# Autodesk Inventor assembly: ASY MSC 100.3 ROСKET NOSE
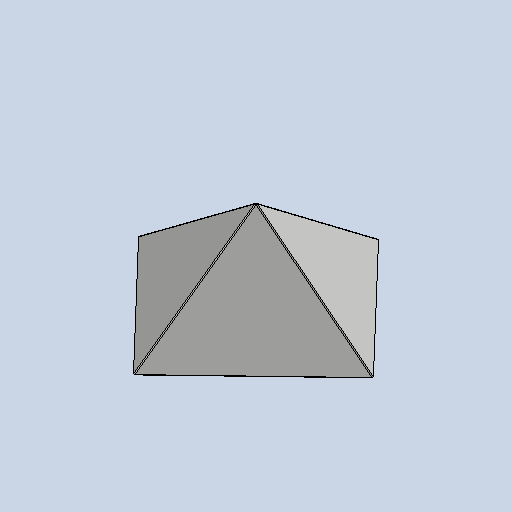
[picture p0: Inventor's stored thumbnail of the model, 512x512]
Saved by Autodesk Inventor 2025 (Build 290162010, 162A)
## iProperties
Created: 2024-09-14
Part Number: ASY MSC 100.3 ROСKET NOSE
Document SubType Name: Assembly
Designer: admin
Author: admin
## Documents named in this file (2)
- C:\Users\admin\YandexDisk-badmisterfox\домашниий пк\Inventor\Manturovo\Manturovo_Se-clar\ASY MSC 100.3 roсket nose.iam
- C:\Users\admin\YandexDisk-badmisterfox\домашниий пк\Inventor\Manturovo\Manturovo_Se-clar\MSC 103 roсket nose.ipt
## Components (4 placed, 1 different names)
1. MSC 103 roсket nose.ipt:1 — Mate:8
2. MSC 103 roсket nose.ipt:2 — Mate:7
3. MSC 103 roсket nose.ipt:3 — Mate:5
4. MSC 103 roсket nose.ipt:4 — Mate:6
## Relationships (8: Mate 8)
- [Mate]: MSC 103 roсket nose.ipt:1 ↔ MSC 103 roсket nose.ipt:3
- [Mate]: MSC 103 roсket nose.ipt:3 ↔ MSC 103 roсket nose.ipt:4
- [Mate]: MSC 103 roсket nose.ipt:2 ↔ MSC 103 roсket nose.ipt:4
- [Mate]: MSC 103 roсket nose.ipt:1 ↔ MSC 103 roсket nose.ipt:2
- Mate:5: MSC 103 roсket nose.ipt:3
- Mate:6: MSC 103 roсket nose.ipt:4
- Mate:7: MSC 103 roсket nose.ipt:2
- Mate:8: MSC 103 roсket nose.ipt:1
